# Autodesk Inventor assembly: LaserFrameAssembly
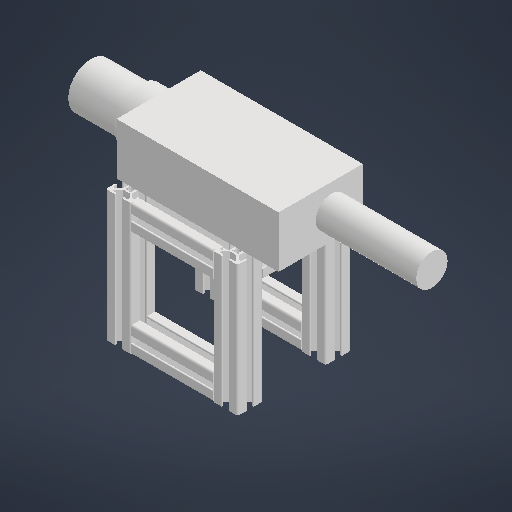
[picture p0: Inventor's stored thumbnail of the model, 512x512]
Saved by Autodesk Inventor 2025 (Build 290162000, 162)
## iProperties
Created: 2024-06-18
Part Number: LaserFrameAssembly
Document SubType Name: Assembly
Designer: mumin
Author: mumin
## Documents named in this file (5)
- C:\Users\mayhe\OneDrive\Documents\GitHub\In-situ-monitoring-of-powder-bed-fusion-additive-manufacturing\system_development\Orichalcum\v0.2\Hardware_design\custom-cover\LaserFrameAssembly.iam
- C:\Users\mayhe\OneDrive\Documents\GitHub\In-situ-monitoring-of-powder-bed-fusion-additive-manufacturing\system_development\Orichalcum\v0.2\Hardware_design\custom-cover\8020-parts\20-2020-104.025.ipt
- C:\Users\mayhe\OneDrive\Documents\GitHub\In-situ-monitoring-of-powder-bed-fusion-additive-manufacturing\system_development\Orichalcum\v0.2\Hardware_design\laser-vibrometer\Updated Laser Scanner.ipt
- C:\Users\mayhe\OneDrive\Documents\GitHub\In-situ-monitoring-of-powder-bed-fusion-additive-manufacturing\system_development\Orichalcum\v0.2\Hardware_design\custom-cover\8020-parts\20-2020-50.ipt
- C:\Users\mayhe\OneDrive\Documents\GitHub\In-situ-monitoring-of-powder-bed-fusion-additive-manufacturing\system_development\Orichalcum\v0.2\Hardware_design\custom-cover\8020-parts\20-2020-65.ipt
## Components (11 placed, 4 different names)
1. 20-2020-50:1 — Mate:1, Flush:1, Flush:2, Mate:6, Flush:11, Flush:12
2. 20-2020-104.025:1 — Mate:1, Flush:1, Flush:2, Mate:2, Flush:3, Flush:4, Mate:3, Flush:5, Flush:6
3. 20-2020-104.025:3 — Mate:4, Flush:7, Flush:8, Mate:5, Flush:9, Flush:10, Mate:6, Flush:11, Flush:12
4. 20-2020-65:1 — Mate:2, Flush:3, Flush:4, Mate:9, Flush:17, Flush:18
5. 20-2020-65:2 — Mate:3, Flush:5, Flush:6
6. 20-2020-65:3 — Mate:4, Flush:7, Flush:8
7. 20-2020-65:4 — Mate:5, Flush:9, Flush:10
8. 20-2020-50:2 — Insert:1
9. 20-2020-104.025:4 — Mate:9, Flush:17, Flush:18
10. 20-2020-104.025:5
11. Updated Laser Scanner:1 — Insert:1
## Relationships (28: Flush 18, Mate 9, Insert 1)
- Mate:1: 20-2020-50:1 ↔ 20-2020-104.025:1
- Flush:1: 20-2020-50:1 ↔ 20-2020-104.025:1
- Flush:2: 20-2020-50:1 ↔ 20-2020-104.025:1
- Mate:2: 20-2020-104.025:1 ↔ 20-2020-65:1
- Flush:3: 20-2020-104.025:1 ↔ 20-2020-65:1
- Flush:4: 20-2020-104.025:1 ↔ 20-2020-65:1
- Mate:3: 20-2020-104.025:1 ↔ 20-2020-65:2
- Flush:5: 20-2020-104.025:1 ↔ 20-2020-65:2
- Flush:6: 20-2020-104.025:1 ↔ 20-2020-65:2
- Mate:4: 20-2020-104.025:3 ↔ 20-2020-65:3
- Flush:7: 20-2020-104.025:3 ↔ 20-2020-65:3
- Flush:8: 20-2020-104.025:3 ↔ 20-2020-65:3
- Mate:5: 20-2020-104.025:3 ↔ 20-2020-65:4
- Flush:9: 20-2020-104.025:3 ↔ 20-2020-65:4
- Flush:10: 20-2020-104.025:3 ↔ 20-2020-65:4
- Mate:6: 20-2020-50:1 ↔ 20-2020-104.025:3
- Flush:11: 20-2020-50:1 ↔ 20-2020-104.025:3
- Flush:12: 20-2020-50:1 ↔ 20-2020-104.025:3
- [Mate]: 20-2020-50:2 ↔ 20-2020-104.025:4
- [Flush]: 20-2020-50:2 ↔ 20-2020-104.025:4
- [Flush]: 20-2020-50:2 ↔ 20-2020-104.025:4
- [Mate]: 20-2020-50:2 ↔ 20-2020-104.025:5
- [Flush]: 20-2020-50:2 ↔ 20-2020-104.025:5
- [Flush]: 20-2020-50:2 ↔ 20-2020-104.025:5
- Mate:9: 20-2020-65:1 ↔ 20-2020-104.025:4
- Flush:17: 20-2020-65:1 ↔ 20-2020-104.025:4
- Flush:18: 20-2020-65:1 ↔ 20-2020-104.025:4
- Insert:1 (6.34 mm): 20-2020-50:2 ↔ Updated Laser Scanner:1
## Named parameters: d43_d2 = 0 mm, d44_d0 = 0 mm, d45_d1 = 0 mm, d46_d40 = 0 mm, d47_d41 = 0 mm, d48_d42 = 0 mm
